# Autodesk Inventor assembly: Assembly
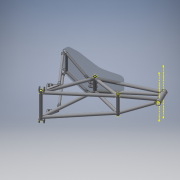
[picture p0: Inventor's stored thumbnail of the model, 180x180]
Saved by Autodesk Inventor 2018 (Build 220112000, 112)
## iProperties
Created: 2018-01-07
Part Number: Assembly
Document SubType Name: Assembly
Designer: eroldan
Author: eroldan
## Documents named in this file (3)
- C:\Users\eroldan\Desktop\3dprojects\OpenEmoto\MainFrame\SeatMount\Assembly.iam
- C:\Users\eroldan\Desktop\3dprojects\OpenEmoto\MainFrame\SeatMount\SeatMount.ipt
- C:\Users\eroldan\Desktop\3dprojects\OpenEmoto\OtherParts\SeatKLX110.ipt
## Components (2 placed, 2 different names)
1. SeatMount:1 — Flush:1, Flush:5
2. SeatKLX110:1 — Flush:6
## Relationships (4: Flush 4)
- Flush:1: SeatMount:1
- Flush:3 (75 mm)
- Flush:5: SeatMount:1
- Flush:6: SeatKLX110:1
